# Autodesk Inventor assembly: Conveyor Module
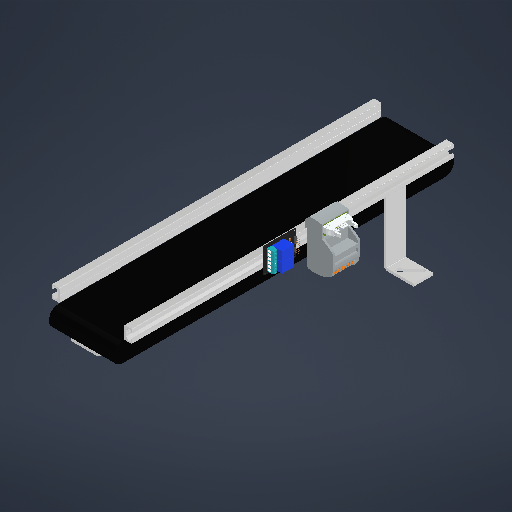
[picture p0: Inventor's stored thumbnail of the model, 512x512]
Saved by Autodesk Inventor 2027 (Build 310192000, 192)
## iProperties
Created: 2026-04-16
Part Number: Conveyor Module
Document SubType Name: Assembly
Designer: ratik
Author: ratik
## Documents named in this file (6)
- C:\Users\ratik\OneDrive\Personal Folder\00_Startup\01_Mectosys_Prototype\01_Prototype\01_Mechanical\3D file\Assembly File\Conveyor Module.iam
- C:\Users\ratik\OneDrive\Personal Folder\00_Startup\01_Mectosys_Prototype\01_Prototype\01_Mechanical\3D file\03_Conveyor Assembly\17_Stainless Steel Mini Conveyor, DC 12 V\Stainless Steel Mini Conveyor, DC 12 V.ipt
- C:\Users\ratik\OneDrive\Personal Folder\00_Startup\01_Mectosys_Prototype\01_Prototype\01_Mechanical\3D file\03_Conveyor Assembly\19_Conveyor mounting bracket\Conveyor mounting bracket.ipt
- C:\Users\ratik\OneDrive\Personal Folder\00_Startup\01_Mectosys_Prototype\01_Prototype\01_Mechanical\3D file\03_Conveyor Assembly\18_Motor controller\2ph63091a-2-channel-5v-relay-module-1.snapshot.2\2PH63091A Pa.ipt
- C:\Users\ratik\OneDrive\Personal Folder\00_Startup\01_Mectosys_Prototype\01_Prototype\01_Mechanical\3D file\02_Slider\08_HFSPURE6-1220-2500_STEP_AP214_20260415\HFSPURE6-1220-2500\HFSPURE6-1220-2500.ipt
- C:\Users\ratik\OneDrive\Personal Folder\00_Startup\01_Mectosys_Prototype\01_Prototype\01_Mechanical\3D file\03_Conveyor Assembly\23_181857052-9-2903801\2903801.ipt
## Components (7 placed, 5 different names)
1. Stainless Steel Mini Conveyor, DC 12 V:1 — Mate:1, Flush:1, Mate:2, Flush:2, Mate:3, Mate:4
2. Conveyor mounting bracket:1 — Mate:1, Flush:1
3. Conveyor mounting bracket:2 — Mate:2, Flush:2
4. 2PH63091A Pa:1 — Mate:5
5. HFSPURE6-1220-2500:1 — Mate:3, Mate:5, Mate:6
6. HFSPURE6-1220-2500:2 — Mate:4
7. 2903801:1 — Mate:6
## Relationships (8: Mate 6, Flush 2)
- Mate:1: Stainless Steel Mini Conveyor, DC 12 V:1 ↔ Conveyor mounting bracket:1
- Flush:1: Stainless Steel Mini Conveyor, DC 12 V:1 ↔ Conveyor mounting bracket:1
- Mate:2: Stainless Steel Mini Conveyor, DC 12 V:1 ↔ Conveyor mounting bracket:2
- Flush:2: Stainless Steel Mini Conveyor, DC 12 V:1 ↔ Conveyor mounting bracket:2
- Mate:3: Stainless Steel Mini Conveyor, DC 12 V:1 ↔ HFSPURE6-1220-2500:1
- Mate:4: Stainless Steel Mini Conveyor, DC 12 V:1 ↔ HFSPURE6-1220-2500:2
- Mate:5: 2PH63091A Pa:1 ↔ HFSPURE6-1220-2500:1
- Mate:6: HFSPURE6-1220-2500:1 ↔ 2903801:1
